# Autodesk Inventor assembly: Selection
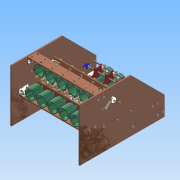
[picture p0: Inventor's stored thumbnail of the model, 180x180]
Saved by Autodesk Inventor 2018.1 (Build 221171000, 171)
## iProperties
Created: 2019-02-07
Part Number: Selection
Document SubType Name: Assembly
Designer: James
Author: James
## Documents named in this file (18)
- C:\Users\admin\Desktop\Ball Sorting Machine\Ball-Sorting-Machine\Prototype CAD\Selection Sort - 40mm\Prototype_Selection Assy 40mm.iam
- C:\Users\admin\Desktop\Ball Sorting Machine\Ball-Sorting-Machine\Prototype CAD\Selection Sort - 40mm\Prototype_LHS.ipt
- C:\Users\admin\Desktop\Ball Sorting Machine\Ball-Sorting-Machine\Prototype CAD\Selection Sort - 40mm\Prototype_Ramp 1.iam
- C:\Users\admin\Desktop\Ball Sorting Machine\Ball-Sorting-Machine\Prototype CAD\Selection Sort - 40mm\SAFL212 Oval 2 Bolt Flanged Unit.ipt
- C:\Users\admin\Desktop\Ball Sorting Machine\Ball-Sorting-Machine\Prototype CAD\Timing Gate - 40mm\Prototype_Timing Assy 40mm.iam
- C:\Users\admin\Desktop\Ball Sorting Machine\Ball-Sorting-Machine\Prototype CAD\Selection Sort - 40mm\Nyloc Nut - M4.ipt
- C:\Users\admin\Desktop\Ball Sorting Machine\Ball-Sorting-Machine\Prototype CAD\Selection Sort - 40mm\Socket Cap Screw - Standard - (A2) - M4 x 16.ipt
- C:\Users\admin\Desktop\Ball Sorting Machine\Ball-Sorting-Machine\Prototype CAD\Selection Sort - 40mm\Locknut - M3.ipt
- C:\Users\admin\Desktop\Ball Sorting Machine\Ball-Sorting-Machine\Prototype CAD\Selection Sort - 40mm\Socket Cap Screw - Standard - (A2) - M3 x 16.ipt
- C:\Users\admin\Desktop\Ball Sorting Machine\Ball-Sorting-Machine\Prototype CAD\Selection Sort - 40mm\Prototype_Exit Pipe Assy.iam
- C:\Users\admin\Desktop\Ball Sorting Machine\Ball-Sorting-Machine\Prototype CAD\Selection Sort - 40mm\Prototype_Shaft Assy.iam
- C:\Users\admin\Desktop\Ball Sorting Machine\Ball-Sorting-Machine\Prototype CAD\Selection Sort - 40mm\Prototype_Lever 1.ipt
- C:\Users\admin\Desktop\Ball Sorting Machine\Ball-Sorting-Machine\Prototype CAD\Selection Sort - 40mm\Socket Cap Screw - Standard - (A2) - M4 x 20.ipt
- C:\Users\admin\Desktop\Ball Sorting Machine\Ball-Sorting-Machine\Prototype CAD\Selection Sort - 40mm\Prototype_Lever Mount Piece.ipt
- C:\Users\admin\Desktop\Ball Sorting Machine\Ball-Sorting-Machine\Prototype CAD\Selection Sort - 40mm\Socket Cap Screw - Standard - (A2) - M3 x 8.ipt
- C:\Users\admin\Desktop\Ball Sorting Machine\Ball-Sorting-Machine\Prototype CAD\Selection Sort - 40mm\Prototype_Washer.ipt
- C:\Users\admin\Desktop\Ball Sorting Machine\Ball-Sorting-Machine\Prototype CAD\Selection Sort - 40mm\Prototype_Lever 3.ipt
- C:\Users\admin\Desktop\Ball Sorting Machine\Ball-Sorting-Machine\Prototype CAD\Selection Sort - 40mm\Ball 40mm.ipt
## Components (92 placed, 17 different names)
1. Prototype_LHS:1 — Flush:1, Flush:2, Flush:3, Mate:4, Flush:9, Flush:10, Mate:37, Mate:38, Mate:39, Mate:42, Mate:43, Mate:56, Mate:70, Mate:71, Mate:116, Mate:117, Mate:118, Mate:119, Mate:120, Mate:121, Mate:128, Mate:129, Mate:131, Mate:152, Mate:155, Mate:193, Mate:194, Mate:195, Mate:196, Mate:200, Mate:203, Mate:204, Mate:205, Mate:206, Mate:207, Mate:208, Mate:210, Mate:211, Mate:213, Mate:214, Mate:225, Mate:226, Mate:227, Mate:228, Mate:232, Mate:233, Mate:234
2. Prototype_Ramp 1:1 [sub-assembly] — Flush:7, Mate:9, Mate:74, Mate:75, Mate:80, Mate:81, Mate:86, Mate:87, Mate:96, Mate:97, Mate:98, Mate:99, Tangent:4
3. Prototype_Ramp 1:2 [sub-assembly] — Mate:4, Mate:76, Mate:77, Mate:82, Mate:83, Mate:88, Mate:89, Mate:94, Mate:95, Mate:102, Mate:103
4. Prototype_Ramp 1:3 [sub-assembly] — Flush:8, Mate:78, Mate:79, Mate:84, Mate:85, Mate:90, Mate:91, Mate:92, Mate:93, Mate:100, Mate:101
5. Prototype_LHS:2 — Mate:9, Flush:9, Flush:10, Mate:52, Mate:53, Mate:54, Mate:55, Mate:57, Mate:62, Mate:63, Mate:74, Mate:75, Mate:76, Mate:77, Mate:78, Mate:79, Mate:104, Mate:105, Mate:106, Mate:107, Mate:108, Mate:109, Mate:132, Mate:134, Mate:135, Mate:148, Mate:149, Mate:159, Mate:160, Mate:161, Mate:162, Mate:163, Mate:164, Mate:189, Mate:190, Mate:191, Mate:192, Mate:197
6. Prototype_Timing Assy 40mm:1 [sub-assembly] — Mate:36, Mate:37, Mate:38, Mate:39, Mate:40, Mate:41, Mate:44, Mate:45, Mate:48, Mate:49, Mate:50, Mate:51, Mate:56, Mate:57, Mate:58, Mate:59, Mate:60, Mate:61, Mate:66, Mate:67, Mate:68, Mate:69
7. SAFL212 Oval 2 Bolt Flanged Unit:3 — Mate:128, Mate:129, Mate:131, Mate:150, Mate:151, Mate:153, Mate:154, Mate:198
8. SAFL212 Oval 2 Bolt Flanged Unit:4 — Mate:132, Mate:134, Mate:135, Mate:144, Mate:145, Mate:146, Mate:147
9. Prototype_Exit Pipe Assy:1 [sub-assembly] — Mate:162, Mate:163, Mate:164, Mate:175, Mate:176, Mate:177, Mate:178, Mate:181, Mate:182, Mate:183, Mate:184
10. Prototype_Exit Pipe Assy:2 [sub-assembly] — Mate:159, Mate:160, Mate:161, Mate:173, Mate:174, Mate:179, Mate:180, Mate:185, Mate:186, Mate:187, Mate:188
11. Prototype_Shaft Assy:1 [sub-assembly] — Mate:197, Flush:11, Mate:198, Tangent:1, Tangent:2, Flush:12
12. Prototype_Lever 1:1 — Mate:200, Flush:12, Mate:209, Mate:212
13. Prototype_Lever Mount Piece:1 — Mate:209, Mate:210, Mate:211, Mate:212, Mate:215, Mate:216, Mate:217
14. Prototype_Washer:1 — Mate:216, Mate:217, Mate:218
15. Prototype_Lever Mount Piece:2 — Mate:226, Mate:228, Mate:229, Mate:230
16. Prototype_Washer:2
17. Prototype_Lever 3:1 — Mate:229, Mate:230, Tangent:3
18. Ball 40mm:1 — Tangent:4
19. Socket Cap Screw - Standard - (A2) - M3 x 8:3 — Mate:225, Mate:227
20. Socket Cap Screw - Standard - (A2) - M3 x 8:4
21. Socket Cap Screw - Standard - (A2) - M3 x 16:9 — Mate:232, Mate:233, Tangent:3
22. Locknut - M3:9 — Mate:234
23. Socket Cap Screw - Standard - (A2) - M3 x 8:2 — Mate:215, Mate:218
24. Socket Cap Screw - Standard - (A2) - M3 x 8:1 — Mate:213, Mate:214
25. Nyloc Nut - M4:25 — Mate:207
26. Socket Cap Screw - Standard - (A2) - M4 x 20:2 — Mate:203, Mate:204, Tangent:1
27. Nyloc Nut - M4:26 — Mate:208
28. Socket Cap Screw - Standard - (A2) - M4 x 20:1 — Mate:205, Mate:206, Tangent:2
29. Nyloc Nut - M4:17 — Mate:173, Mate:179
30. Socket Cap Screw - Standard - (A2) - M4 x 16:17 — Mate:195
31. Nyloc Nut - M4:18 — Mate:174, Mate:180
32. Socket Cap Screw - Standard - (A2) - M4 x 16:18 — Mate:196
33. Nyloc Nut - M4:19 — Mate:175, Mate:176
34. Socket Cap Screw - Standard - (A2) - M4 x 16:19 — Mate:193
35. Nyloc Nut - M4:20 — Mate:177, Mate:178
36. Socket Cap Screw - Standard - (A2) - M4 x 16:20 — Mate:194
37. Nyloc Nut - M4:21 — Mate:181, Mate:183
38. Socket Cap Screw - Standard - (A2) - M4 x 16:21 — Mate:189
39. Nyloc Nut - M4:22 — Mate:182, Mate:184
40. Socket Cap Screw - Standard - (A2) - M4 x 16:22 — Mate:190
41. Nyloc Nut - M4:23 — Mate:185, Mate:188
42. Socket Cap Screw - Standard - (A2) - M4 x 16:23 — Mate:192
43. Nyloc Nut - M4:24 — Mate:186, Mate:187
44. Socket Cap Screw - Standard - (A2) - M4 x 16:24 — Mate:191
45. Locknut - M3:5 — Mate:149
46. Socket Cap Screw - Standard - (A2) - M3 x 16:5 — Mate:144, Mate:145
47. Locknut - M3:6 — Mate:148
48. Socket Cap Screw - Standard - (A2) - M3 x 16:6 — Mate:146, Mate:147
49. Locknut - M3:7 — Mate:152
50. Socket Cap Screw - Standard - (A2) - M3 x 16:7 — Mate:150, Mate:151
51. Locknut - M3:8 — Mate:155
52. Socket Cap Screw - Standard - (A2) - M3 x 16:8 — Mate:153, Mate:154
53. Nyloc Nut - M4:1 — Mate:44, Mate:46
54. Socket Cap Screw - Standard - (A2) - M4 x 16:1 — Mate:41, Mate:43, Mate:47
55. Nyloc Nut - M4:2 — Mate:45, Mate:47
56. Socket Cap Screw - Standard - (A2) - M4 x 16:2 — Mate:40, Mate:42, Mate:46
57. Nyloc Nut - M4:3 — Mate:49, Mate:50
58. Socket Cap Screw - Standard - (A2) - M4 x 16:3 — Mate:53, Mate:54
59. Nyloc Nut - M4:4 — Mate:48, Mate:51
60. Socket Cap Screw - Standard - (A2) - M4 x 16:4 — Mate:52, Mate:55
61. Locknut - M3:1 — Mate:62, Mate:64
62. Socket Cap Screw - Standard - (A2) - M3 x 16:1 — Mate:58, Mate:60, Mate:64
63. Locknut - M3:2 — Mate:63, Mate:65
64. Socket Cap Screw - Standard - (A2) - M3 x 16:2 — Mate:59, Mate:61, Mate:65
65. Locknut - M3:3 — Mate:70, Mate:72
66. Socket Cap Screw - Standard - (A2) - M3 x 16:3 — Mate:66, Mate:67, Mate:72
67. Locknut - M3:4 — Mate:71, Mate:73
68. Socket Cap Screw - Standard - (A2) - M3 x 16:4 — Mate:68, Mate:69, Mate:73
69. Nyloc Nut - M4:5 — Mate:104, Mate:110
70. Socket Cap Screw - Standard - (A2) - M4 x 16:5 — Mate:80, Mate:98, Mate:110
71. Nyloc Nut - M4:6 — Mate:105, Mate:112
72. Socket Cap Screw - Standard - (A2) - M4 x 16:6 — Mate:82, Mate:103, Mate:112
73. Nyloc Nut - M4:7 — Mate:106, Mate:115
74. Socket Cap Screw - Standard - (A2) - M4 x 16:7 — Mate:83, Mate:102, Mate:113
75. Nyloc Nut - M4:8 — Mate:107, Mate:113
76. Socket Cap Screw - Standard - (A2) - M4 x 16:8 — Mate:84, Mate:101, Mate:115
77. Nyloc Nut - M4:9 — Mate:108, Mate:111
78. Socket Cap Screw - Standard - (A2) - M4 x 16:9 — Mate:90, Mate:92, Mate:125
79. Nyloc Nut - M4:10 — Mate:109, Mate:114
80. Socket Cap Screw - Standard - (A2) - M4 x 16:10 — Mate:85, Mate:100, Mate:114
81. Nyloc Nut - M4:11 — Mate:116, Mate:124
82. Socket Cap Screw - Standard - (A2) - M4 x 16:11 — Mate:81, Mate:99, Mate:111
83. Nyloc Nut - M4:12 — Mate:117, Mate:126
84. Socket Cap Screw - Standard - (A2) - M4 x 16:12 — Mate:86, Mate:96, Mate:122
85. Nyloc Nut - M4:13 — Mate:118, Mate:127
86. Socket Cap Screw - Standard - (A2) - M4 x 16:13 — Mate:87, Mate:97, Mate:124
87. Nyloc Nut - M4:14 — Mate:119, Mate:125
88. Socket Cap Screw - Standard - (A2) - M4 x 16:14 — Mate:88, Mate:95, Mate:123
89. Nyloc Nut - M4:15 — Mate:120, Mate:123
90. Socket Cap Screw - Standard - (A2) - M4 x 16:15 — Mate:89, Mate:94, Mate:127
91. Nyloc Nut - M4:16 — Mate:121, Mate:122
92. Socket Cap Screw - Standard - (A2) - M4 x 16:16 — Mate:91, Mate:93, Mate:126
## Relationships (202: Mate 189, Flush 9, Tangent 4)
- Flush:1: Prototype_LHS:1
- Flush:2: Prototype_LHS:1
- Flush:3: Prototype_LHS:1
- Flush:7: Prototype_Ramp 1:1
- Mate:4: Prototype_LHS:1 ↔ Prototype_Ramp 1:2
- Flush:8: Prototype_Ramp 1:3
- Mate:9: Prototype_Ramp 1:1 ↔ Prototype_LHS:2
- Flush:9: Prototype_LHS:1 ↔ Prototype_LHS:2
- Flush:10: Prototype_LHS:1 ↔ Prototype_LHS:2
- Mate:36: Prototype_Timing Assy 40mm:1
- Mate:37: Prototype_LHS:1 ↔ Prototype_Timing Assy 40mm:1
- Mate:38: Prototype_LHS:1 ↔ Prototype_Timing Assy 40mm:1
- Mate:39: Prototype_LHS:1 ↔ Prototype_Timing Assy 40mm:1
- Mate:40: Prototype_Timing Assy 40mm:1 ↔ Socket Cap Screw - Standard - (A2) - M4 x 16:2
- Mate:41: Prototype_Timing Assy 40mm:1 ↔ Socket Cap Screw - Standard - (A2) - M4 x 16:1
- Mate:42: Prototype_LHS:1 ↔ Socket Cap Screw - Standard - (A2) - M4 x 16:2
- Mate:43: Prototype_LHS:1 ↔ Socket Cap Screw - Standard - (A2) - M4 x 16:1
- Mate:44: Prototype_Timing Assy 40mm:1 ↔ Nyloc Nut - M4:1
- Mate:45: Prototype_Timing Assy 40mm:1 ↔ Nyloc Nut - M4:2
- Mate:46: Nyloc Nut - M4:1 ↔ Socket Cap Screw - Standard - (A2) - M4 x 16:2
- Mate:47: Socket Cap Screw - Standard - (A2) - M4 x 16:1 ↔ Nyloc Nut - M4:2
- Mate:48: Prototype_Timing Assy 40mm:1 ↔ Nyloc Nut - M4:4
- Mate:49: Prototype_Timing Assy 40mm:1 ↔ Nyloc Nut - M4:3
- Mate:50: Prototype_Timing Assy 40mm:1 ↔ Nyloc Nut - M4:3
- Mate:51: Prototype_Timing Assy 40mm:1 ↔ Nyloc Nut - M4:4
- Mate:52: Prototype_LHS:2 ↔ Socket Cap Screw - Standard - (A2) - M4 x 16:4
- Mate:53: Prototype_LHS:2 ↔ Socket Cap Screw - Standard - (A2) - M4 x 16:3
- Mate:54: Prototype_LHS:2 ↔ Socket Cap Screw - Standard - (A2) - M4 x 16:3
- Mate:55: Prototype_LHS:2 ↔ Socket Cap Screw - Standard - (A2) - M4 x 16:4
- Mate:56: Prototype_LHS:1 ↔ Prototype_Timing Assy 40mm:1
- Mate:57: Prototype_LHS:2 ↔ Prototype_Timing Assy 40mm:1
- Mate:58: Prototype_Timing Assy 40mm:1 ↔ Socket Cap Screw - Standard - (A2) - M3 x 16:1
- Mate:59: Prototype_Timing Assy 40mm:1 ↔ Socket Cap Screw - Standard - (A2) - M3 x 16:2
- Mate:60: Prototype_Timing Assy 40mm:1 ↔ Socket Cap Screw - Standard - (A2) - M3 x 16:1
- Mate:61: Prototype_Timing Assy 40mm:1 ↔ Socket Cap Screw - Standard - (A2) - M3 x 16:2
- Mate:62: Prototype_LHS:2 ↔ Locknut - M3:1
- Mate:63: Prototype_LHS:2 ↔ Locknut - M3:2
- Mate:64: Locknut - M3:1 ↔ Socket Cap Screw - Standard - (A2) - M3 x 16:1
- Mate:65: Locknut - M3:2 ↔ Socket Cap Screw - Standard - (A2) - M3 x 16:2
- Mate:66: Prototype_Timing Assy 40mm:1 ↔ Socket Cap Screw - Standard - (A2) - M3 x 16:3
- Mate:67: Prototype_Timing Assy 40mm:1 ↔ Socket Cap Screw - Standard - (A2) - M3 x 16:3
- Mate:68: Prototype_Timing Assy 40mm:1 ↔ Socket Cap Screw - Standard - (A2) - M3 x 16:4
- Mate:69: Prototype_Timing Assy 40mm:1 ↔ Socket Cap Screw - Standard - (A2) - M3 x 16:4
- Mate:70: Prototype_LHS:1 ↔ Locknut - M3:3
- Mate:71: Prototype_LHS:1 ↔ Locknut - M3:4
- Mate:72: Locknut - M3:3 ↔ Socket Cap Screw - Standard - (A2) - M3 x 16:3
- Mate:73: Locknut - M3:4 ↔ Socket Cap Screw - Standard - (A2) - M3 x 16:4
- Mate:74: Prototype_Ramp 1:1 ↔ Prototype_LHS:2
- Mate:75: Prototype_Ramp 1:1 ↔ Prototype_LHS:2
- Mate:76: Prototype_Ramp 1:2 ↔ Prototype_LHS:2
- Mate:77: Prototype_Ramp 1:2 ↔ Prototype_LHS:2
- Mate:78: Prototype_Ramp 1:3 ↔ Prototype_LHS:2
- Mate:79: Prototype_Ramp 1:3 ↔ Prototype_LHS:2
- Mate:80: Prototype_Ramp 1:1 ↔ Socket Cap Screw - Standard - (A2) - M4 x 16:5
- Mate:81: Prototype_Ramp 1:1 ↔ Socket Cap Screw - Standard - (A2) - M4 x 16:11
- Mate:82: Prototype_Ramp 1:2 ↔ Socket Cap Screw - Standard - (A2) - M4 x 16:6
- Mate:83: Prototype_Ramp 1:2 ↔ Socket Cap Screw - Standard - (A2) - M4 x 16:7
- Mate:84: Prototype_Ramp 1:3 ↔ Socket Cap Screw - Standard - (A2) - M4 x 16:8
- Mate:85: Prototype_Ramp 1:3 ↔ Socket Cap Screw - Standard - (A2) - M4 x 16:10
- Mate:86: Prototype_Ramp 1:1 ↔ Socket Cap Screw - Standard - (A2) - M4 x 16:12
- Mate:87: Prototype_Ramp 1:1 ↔ Socket Cap Screw - Standard - (A2) - M4 x 16:13
- Mate:88: Prototype_Ramp 1:2 ↔ Socket Cap Screw - Standard - (A2) - M4 x 16:14
- Mate:89: Prototype_Ramp 1:2 ↔ Socket Cap Screw - Standard - (A2) - M4 x 16:15
- Mate:90: Prototype_Ramp 1:3 ↔ Socket Cap Screw - Standard - (A2) - M4 x 16:9
- Mate:91: Prototype_Ramp 1:3 ↔ Socket Cap Screw - Standard - (A2) - M4 x 16:16
- Mate:92: Prototype_Ramp 1:3 ↔ Socket Cap Screw - Standard - (A2) - M4 x 16:9
- Mate:93: Prototype_Ramp 1:3 ↔ Socket Cap Screw - Standard - (A2) - M4 x 16:16
- Mate:94: Prototype_Ramp 1:2 ↔ Socket Cap Screw - Standard - (A2) - M4 x 16:15
- Mate:95: Prototype_Ramp 1:2 ↔ Socket Cap Screw - Standard - (A2) - M4 x 16:14
- Mate:96: Prototype_Ramp 1:1 ↔ Socket Cap Screw - Standard - (A2) - M4 x 16:12
- Mate:97: Prototype_Ramp 1:1 ↔ Socket Cap Screw - Standard - (A2) - M4 x 16:13
- Mate:98: Prototype_Ramp 1:1 ↔ Socket Cap Screw - Standard - (A2) - M4 x 16:5
- Mate:99: Prototype_Ramp 1:1 ↔ Socket Cap Screw - Standard - (A2) - M4 x 16:11
- Mate:100: Prototype_Ramp 1:3 ↔ Socket Cap Screw - Standard - (A2) - M4 x 16:10
- Mate:101: Prototype_Ramp 1:3 ↔ Socket Cap Screw - Standard - (A2) - M4 x 16:8
- Mate:102: Prototype_Ramp 1:2 ↔ Socket Cap Screw - Standard - (A2) - M4 x 16:7
- Mate:103: Prototype_Ramp 1:2 ↔ Socket Cap Screw - Standard - (A2) - M4 x 16:6
- Mate:104: Prototype_LHS:2 ↔ Nyloc Nut - M4:5
- Mate:105: Prototype_LHS:2 ↔ Nyloc Nut - M4:6
- Mate:106: Prototype_LHS:2 ↔ Nyloc Nut - M4:7
- Mate:107: Prototype_LHS:2 ↔ Nyloc Nut - M4:8
- Mate:108: Prototype_LHS:2 ↔ Nyloc Nut - M4:9
- Mate:109: Prototype_LHS:2 ↔ Nyloc Nut - M4:10
- Mate:110: Nyloc Nut - M4:5 ↔ Socket Cap Screw - Standard - (A2) - M4 x 16:5
- Mate:111: Nyloc Nut - M4:9 ↔ Socket Cap Screw - Standard - (A2) - M4 x 16:11
- Mate:112: Nyloc Nut - M4:6 ↔ Socket Cap Screw - Standard - (A2) - M4 x 16:6
- Mate:113: Socket Cap Screw - Standard - (A2) - M4 x 16:7 ↔ Nyloc Nut - M4:8
- Mate:114: Nyloc Nut - M4:10 ↔ Socket Cap Screw - Standard - (A2) - M4 x 16:10
- Mate:115: Nyloc Nut - M4:7 ↔ Socket Cap Screw - Standard - (A2) - M4 x 16:8
- Mate:116: Prototype_LHS:1 ↔ Nyloc Nut - M4:11
- Mate:117: Prototype_LHS:1 ↔ Nyloc Nut - M4:12
- Mate:118: Prototype_LHS:1 ↔ Nyloc Nut - M4:13
- Mate:119: Prototype_LHS:1 ↔ Nyloc Nut - M4:14
- Mate:120: Prototype_LHS:1 ↔ Nyloc Nut - M4:15
- Mate:121: Prototype_LHS:1 ↔ Nyloc Nut - M4:16
- Mate:122: Socket Cap Screw - Standard - (A2) - M4 x 16:12 ↔ Nyloc Nut - M4:16
- Mate:123: Socket Cap Screw - Standard - (A2) - M4 x 16:14 ↔ Nyloc Nut - M4:15
- Mate:124: Nyloc Nut - M4:11 ↔ Socket Cap Screw - Standard - (A2) - M4 x 16:13
- Mate:125: Socket Cap Screw - Standard - (A2) - M4 x 16:9 ↔ Nyloc Nut - M4:14
- Mate:126: Nyloc Nut - M4:12 ↔ Socket Cap Screw - Standard - (A2) - M4 x 16:16
- Mate:127: Nyloc Nut - M4:13 ↔ Socket Cap Screw - Standard - (A2) - M4 x 16:15
- Mate:128: Prototype_LHS:1 ↔ SAFL212 Oval 2 Bolt Flanged Unit:3
- Mate:129: Prototype_LHS:1 ↔ SAFL212 Oval 2 Bolt Flanged Unit:3
- Mate:131: Prototype_LHS:1 ↔ SAFL212 Oval 2 Bolt Flanged Unit:3
- Mate:132: Prototype_LHS:2 ↔ SAFL212 Oval 2 Bolt Flanged Unit:4
- Mate:134: Prototype_LHS:2 ↔ SAFL212 Oval 2 Bolt Flanged Unit:4
- Mate:135: Prototype_LHS:2 ↔ SAFL212 Oval 2 Bolt Flanged Unit:4
- [Mate]: Locknut - M3:5 ↔ Socket Cap Screw - Standard - (A2) - M3 x 16:5
- [Mate]: Locknut - M3:6 ↔ Socket Cap Screw - Standard - (A2) - M3 x 16:6
- [Mate]: Locknut - M3:7 ↔ Socket Cap Screw - Standard - (A2) - M3 x 16:7
- [Mate]: Locknut - M3:8 ↔ Socket Cap Screw - Standard - (A2) - M3 x 16:8
- Mate:144: SAFL212 Oval 2 Bolt Flanged Unit:4 ↔ Socket Cap Screw - Standard - (A2) - M3 x 16:5
- Mate:145: SAFL212 Oval 2 Bolt Flanged Unit:4 ↔ Socket Cap Screw - Standard - (A2) - M3 x 16:5
- Mate:146: SAFL212 Oval 2 Bolt Flanged Unit:4 ↔ Socket Cap Screw - Standard - (A2) - M3 x 16:6
- Mate:147: SAFL212 Oval 2 Bolt Flanged Unit:4 ↔ Socket Cap Screw - Standard - (A2) - M3 x 16:6
- Mate:148: Prototype_LHS:2 ↔ Locknut - M3:6
- Mate:149: Prototype_LHS:2 ↔ Locknut - M3:5
- Mate:150: SAFL212 Oval 2 Bolt Flanged Unit:3 ↔ Socket Cap Screw - Standard - (A2) - M3 x 16:7
- Mate:151: SAFL212 Oval 2 Bolt Flanged Unit:3 ↔ Socket Cap Screw - Standard - (A2) - M3 x 16:7
- Mate:152: Prototype_LHS:1 ↔ Locknut - M3:7
- Mate:153: SAFL212 Oval 2 Bolt Flanged Unit:3 ↔ Socket Cap Screw - Standard - (A2) - M3 x 16:8
- Mate:154: SAFL212 Oval 2 Bolt Flanged Unit:3 ↔ Socket Cap Screw - Standard - (A2) - M3 x 16:8
- Mate:155: Prototype_LHS:1 ↔ Locknut - M3:8
- Mate:159: Prototype_LHS:2 ↔ Prototype_Exit Pipe Assy:2
- Mate:160: Prototype_LHS:2 ↔ Prototype_Exit Pipe Assy:2
- Mate:161: Prototype_LHS:2 ↔ Prototype_Exit Pipe Assy:2
- Mate:162: Prototype_LHS:2 ↔ Prototype_Exit Pipe Assy:1
- Mate:163: Prototype_LHS:2 ↔ Prototype_Exit Pipe Assy:1
- Mate:164: Prototype_LHS:2 ↔ Prototype_Exit Pipe Assy:1
- [Mate]: Nyloc Nut - M4:17 ↔ Socket Cap Screw - Standard - (A2) - M4 x 16:17
- [Mate]: Nyloc Nut - M4:18 ↔ Socket Cap Screw - Standard - (A2) - M4 x 16:18
- [Mate]: Nyloc Nut - M4:19 ↔ Socket Cap Screw - Standard - (A2) - M4 x 16:19
- [Mate]: Nyloc Nut - M4:20 ↔ Socket Cap Screw - Standard - (A2) - M4 x 16:20
- [Mate]: Nyloc Nut - M4:21 ↔ Socket Cap Screw - Standard - (A2) - M4 x 16:21
- [Mate]: Nyloc Nut - M4:22 ↔ Socket Cap Screw - Standard - (A2) - M4 x 16:22
- [Mate]: Nyloc Nut - M4:23 ↔ Socket Cap Screw - Standard - (A2) - M4 x 16:23
- [Mate]: Nyloc Nut - M4:24 ↔ Socket Cap Screw - Standard - (A2) - M4 x 16:24
- Mate:173: Prototype_Exit Pipe Assy:2 ↔ Nyloc Nut - M4:17
- Mate:174: Prototype_Exit Pipe Assy:2 ↔ Nyloc Nut - M4:18
- Mate:175: Prototype_Exit Pipe Assy:1 ↔ Nyloc Nut - M4:19
- Mate:176: Prototype_Exit Pipe Assy:1 ↔ Nyloc Nut - M4:19
- Mate:177: Prototype_Exit Pipe Assy:1 ↔ Nyloc Nut - M4:20
- Mate:178: Prototype_Exit Pipe Assy:1 ↔ Nyloc Nut - M4:20
- Mate:179: Prototype_Exit Pipe Assy:2 ↔ Nyloc Nut - M4:17
- Mate:180: Prototype_Exit Pipe Assy:2 ↔ Nyloc Nut - M4:18
- Mate:181: Prototype_Exit Pipe Assy:1 ↔ Nyloc Nut - M4:21
- Mate:182: Prototype_Exit Pipe Assy:1 ↔ Nyloc Nut - M4:22
- Mate:183: Prototype_Exit Pipe Assy:1 ↔ Nyloc Nut - M4:21
- Mate:184: Prototype_Exit Pipe Assy:1 ↔ Nyloc Nut - M4:22
- Mate:185: Prototype_Exit Pipe Assy:2 ↔ Nyloc Nut - M4:23
- Mate:186: Prototype_Exit Pipe Assy:2 ↔ Nyloc Nut - M4:24
- Mate:187: Prototype_Exit Pipe Assy:2 ↔ Nyloc Nut - M4:24
- Mate:188: Prototype_Exit Pipe Assy:2 ↔ Nyloc Nut - M4:23
- Mate:189: Prototype_LHS:2 ↔ Socket Cap Screw - Standard - (A2) - M4 x 16:21
- Mate:190: Prototype_LHS:2 ↔ Socket Cap Screw - Standard - (A2) - M4 x 16:22
- Mate:191: Prototype_LHS:2 ↔ Socket Cap Screw - Standard - (A2) - M4 x 16:24
- Mate:192: Prototype_LHS:2 ↔ Socket Cap Screw - Standard - (A2) - M4 x 16:23
- Mate:193: Prototype_LHS:1 ↔ Socket Cap Screw - Standard - (A2) - M4 x 16:19
- Mate:194: Prototype_LHS:1 ↔ Socket Cap Screw - Standard - (A2) - M4 x 16:20
- Mate:195: Prototype_LHS:1 ↔ Socket Cap Screw - Standard - (A2) - M4 x 16:17
- Mate:196: Prototype_LHS:1 ↔ Socket Cap Screw - Standard - (A2) - M4 x 16:18
- Mate:197: Prototype_LHS:2 ↔ Prototype_Shaft Assy:1
- Flush:11: Prototype_Shaft Assy:1
- Mate:198: SAFL212 Oval 2 Bolt Flanged Unit:3 ↔ Prototype_Shaft Assy:1
- Mate:200: Prototype_LHS:1 ↔ Prototype_Lever 1:1
- [Mate]: Nyloc Nut - M4:25 ↔ Socket Cap Screw - Standard - (A2) - M4 x 20:2
- [Mate]: Nyloc Nut - M4:26 ↔ Socket Cap Screw - Standard - (A2) - M4 x 20:1
- Mate:203: Prototype_LHS:1 ↔ Socket Cap Screw - Standard - (A2) - M4 x 20:2
- Mate:204: Prototype_LHS:1 ↔ Socket Cap Screw - Standard - (A2) - M4 x 20:2
- Mate:205: Prototype_LHS:1 ↔ Socket Cap Screw - Standard - (A2) - M4 x 20:1
- Mate:206: Prototype_LHS:1 ↔ Socket Cap Screw - Standard - (A2) - M4 x 20:1
- Mate:207: Prototype_LHS:1 ↔ Nyloc Nut - M4:25
- Mate:208: Prototype_LHS:1 ↔ Nyloc Nut - M4:26
- Tangent:1: Prototype_Shaft Assy:1 ↔ Socket Cap Screw - Standard - (A2) - M4 x 20:2
- Tangent:2: Prototype_Shaft Assy:1 ↔ Socket Cap Screw - Standard - (A2) - M4 x 20:1
- Flush:12: Prototype_Shaft Assy:1 ↔ Prototype_Lever 1:1
- Mate:209: Prototype_Lever 1:1 ↔ Prototype_Lever Mount Piece:1
- Mate:210: Prototype_LHS:1 ↔ Prototype_Lever Mount Piece:1
- Mate:211: Prototype_LHS:1 ↔ Prototype_Lever Mount Piece:1
- Mate:212 (0.5 mm): Prototype_Lever 1:1 ↔ Prototype_Lever Mount Piece:1
- Mate:213: Prototype_LHS:1 ↔ Socket Cap Screw - Standard - (A2) - M3 x 8:1
- Mate:214: Prototype_LHS:1 ↔ Socket Cap Screw - Standard - (A2) - M3 x 8:1
- Mate:215: Prototype_Lever Mount Piece:1 ↔ Socket Cap Screw - Standard - (A2) - M3 x 8:2
- Mate:216: Prototype_Lever Mount Piece:1 ↔ Prototype_Washer:1
- Mate:217: Prototype_Lever Mount Piece:1 ↔ Prototype_Washer:1
- Mate:218: Prototype_Washer:1 ↔ Socket Cap Screw - Standard - (A2) - M3 x 8:2
- [Mate]: Prototype_Lever Mount Piece:2 ↔ Socket Cap Screw - Standard - (A2) - M3 x 8:4
- [Mate]: Prototype_Lever Mount Piece:2 ↔ Prototype_Washer:2
- [Mate]: Prototype_Lever Mount Piece:2 ↔ Prototype_Washer:2
- [Mate]: Prototype_Washer:2 ↔ Socket Cap Screw - Standard - (A2) - M3 x 8:4
- Mate:225: Prototype_LHS:1 ↔ Socket Cap Screw - Standard - (A2) - M3 x 8:3
- Mate:226: Prototype_LHS:1 ↔ Prototype_Lever Mount Piece:2
- Mate:227: Prototype_LHS:1 ↔ Socket Cap Screw - Standard - (A2) - M3 x 8:3
- Mate:228: Prototype_LHS:1 ↔ Prototype_Lever Mount Piece:2
- Mate:229: Prototype_Lever Mount Piece:2 ↔ Prototype_Lever 3:1
- Mate:230: Prototype_Lever Mount Piece:2 ↔ Prototype_Lever 3:1
- [Mate]: Socket Cap Screw - Standard - (A2) - M3 x 16:9 ↔ Locknut - M3:9
- Mate:232: Prototype_LHS:1 ↔ Socket Cap Screw - Standard - (A2) - M3 x 16:9
- Mate:233: Prototype_LHS:1 ↔ Socket Cap Screw - Standard - (A2) - M3 x 16:9
- Mate:234: Prototype_LHS:1 ↔ Locknut - M3:9
- Tangent:3: Prototype_Lever 3:1 ↔ Socket Cap Screw - Standard - (A2) - M3 x 16:9
- Tangent:4: Prototype_Ramp 1:1 ↔ Ball 40mm:1
## Named parameters: d159_d87 = 0 mm, d160_d87 = 0 mm, d161_d87 = 0 mm, d162_d87 = 0 mm, d190_d69 = 0 mm, d191_d69 = 0 mm, d192_d69 = 0 mm, d193_d69 = 0 mm, d194_d69 = 0 mm, d195_d69 = 0 mm, d196_d69 = 0 mm, d197_d69 = 0 mm, d227_d196_d69 = 0 mm, d228_d196_d69 = 0 mm, d254_d248 = 0 mm, d255_d249 = 0 mm, d256_d250 = 0 mm, d257_d251 = 0 mm, d264_d159_d87 = 0 mm
